# Autodesk Inventor assembly: U.FL Female Jack to SMA Female Jack Bulkhead RF Connector
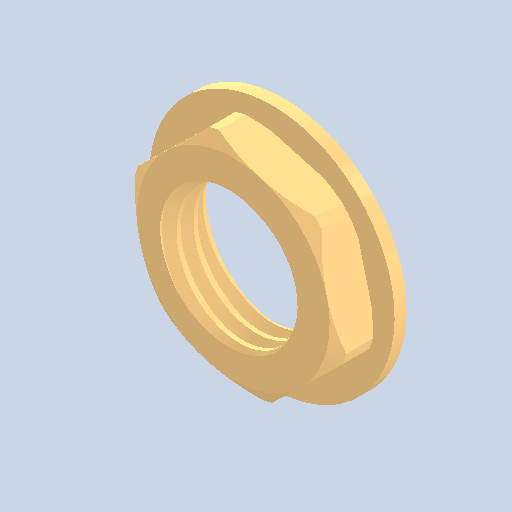
[picture p0: Inventor's stored thumbnail of the model, 512x512]
Saved by Autodesk Inventor 2023.1 (Build 271208000, 208)
## iProperties
Created: 2021-08-18
Part Number: U.FL Female Jack to SMA Female Jack Bulkhead RF Connector
Description: STEP AP214
Document SubType Name: Assembly
Designer: pd
Sending System: SolidWorks 2018
Preprocessor: SwSTEP 2.0
Title: U.FL Female Jack to SMA Female Jack Bulkhead RF Connector.STEP
Revision Number: ANY
## Documents named in this file (3)
- D:\OneDrive\Elektronikprojekte\DAQ v3 STM32H7\CAD\Misc\SMA_Washer_Nut.iam
- D:\OneDrive\Elektronikprojekte\DAQ v3 STM32H7\CAD\Misc\SMA_Washer.ipt
- D:\OneDrive\Elektronikprojekte\DAQ v3 STM32H7\CAD\Misc\SMA_Nut.ipt
## Components (2 placed, 2 different names)
1. SMA_Washer — Passend:1, Passend:2
2. SMA_Nut — Passend:1, Passend:2
## Relationships (2: Mate 2)
- Passend:1 [Mate]: SMA_Washer ↔ SMA_Nut
- Passend:2 [Mate]: SMA_Washer ↔ SMA_Nut
